# Autodesk Inventor assembly: Robot
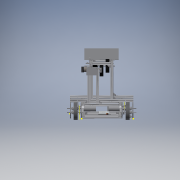
[picture p0: Inventor's stored thumbnail of the model, 180x180]
Saved by Autodesk Inventor 2016 (Build 200138000, 138)
## iProperties
Created: 2016-10-08
Part Number: Robot
Document SubType Name: Assembly
Designer: RoboticsUser
Author: RoboticsUser
## Documents named in this file (17)
- C:\Robotics\CAD\2016-17_CAD\Robot.iam
- C:\Robotics\CAD\2016-17_CAD\WheelAssemblyWFrame.iam
- C:\Robotics\CAD\COTSParts\Bosch Extrusion\Bosch 20x20 9 in.ipt
- C:\Robotics\CAD\COTSParts\Bosch Extrusion\Gusset 20x20 w screws.ipt
- C:\Robotics\CAD\COTSParts\Bosch Extrusion\Bosch 20x20 9 in - Copy.ipt
- C:\Robotics\CAD\COTSParts\Bosch Extrusion\Rexroth-6mmT-Nutm4.ipt
- C:\Robotics\CAD\COTSParts\Bosch Extrusion\Rexroth-GussetwFastenersm4x8.ipt
- C:\Robotics\CAD\COTSParts\Bosch Extrusion\Bosch 20x20 8.937in.ipt
- C:\Robotics\CAD\COTSParts\Bosch Extrusion\Bosch 20x20 9 in actual.ipt
- C:\Robotics\CAD\2016-17_CAD\ParticleLauncher2.0.iam
- C:\Robotics\CAD\2016-17_CAD\BBP.iam
- C:\Robotics\CAD\2016-17_CAD\ElectronicsPlate2.ipt
- C:\Robotics\CAD\COTSParts\ModernRobotics\MRI45-2204_Servo_Controller.ipt
- C:\Robotics\CAD\COTSParts\ModernRobotics\MRI45-2201_Device_Interface.ipt
- C:\Robotics\CAD\2016-17_CAD\Deflecter.ipt
- C:\Robotics\CAD\COTSParts\Bosch Extrusion\Bosch 20x20 16.66 -.ipt
- C:\Robotics\CAD\COTSParts\Actobotics\585 parts\585424.ipt
## Components (55 placed, 16 different names)
1. WheelAssemblyWFrame:1 [sub-assembly] — Mate:1, Insert:4, Insert:5, Insert:6, Flush:29, Mate:55, Flush:37, Flush:42, Flush:83, Mate:144
2. WheelAssemblyWFrame:2 [sub-assembly] — Mate:8, Mate:9, Flush:7, Flush:8, Insert:1, Insert:2, Insert:3, Flush:30, Flush:35, Mate:57, Mate:58, Mate:77, Mate:107, Flush:82, Mate:143, Flush:88, Flush:90, Flush:99
3. Bosch 20x20 9 in:1 — Flush:37, Mate:56, Mate:58, Mate:69, Flush:40, Mate:70, Mate:71, Mate:72, Flush:42, Mate:73, Flush:43, Mate:75, Flush:44, Mate:77
4. Gusset 20x20 w screws:1 — Mate:9, Flush:7, Mate:10
5. Gusset 20x20 w screws:2 — Mate:1
6. Gusset 20x20 w screws:3 — Mate:8
7. Gusset 20x20 w screws:4 — Mate:11, Flush:9
8. Bosch 20x20 9 in:2 — Mate:10, Flush:8, Mate:11, Flush:9, Flush:35, Mate:55
9. Bosch 20x20 9 in - Copy:1 — Mate:33, Flush:25, Flush:28, Flush:30, Flush:31, Mate:44, Flush:34, Mate:52, Mate:53, Mate:131, Mate:142
10. Rexroth-6mmT-Nutm4:1 — Insert:1
11. Rexroth-6mmT-Nutm4:2 — Insert:3, Mate:33, Flush:25
12. Rexroth-6mmT-Nutm4:3 — Insert:2
13. Bosch 20x20 9 in - Copy:2 — Mate:15, Flush:11, Mate:35, Mate:39, Flush:27, Flush:29, Flush:32, Mate:48, Flush:33, Mate:54
14. Rexroth-6mmT-Nutm4:4 — Insert:4
15. Rexroth-6mmT-Nutm4:5 — Insert:5
16. Rexroth-6mmT-Nutm4:6 — Insert:6, Mate:15, Flush:11
17. Bosch 20x20 9 in:3 — Flush:27, Flush:31, Mate:50, Mate:51, Mate:53, Mate:54, Flush:69, Mate:141
18. Bosch 20x20 9 in:4 — Mate:39, Flush:28, Flush:32, Mate:45, Mate:46, Mate:47, Mate:49, Flush:33, Flush:34, Mate:106, Mate:130
19. Gusset 20x20 w screws:5 — Mate:51, Mate:52
20. Gusset 20x20 w screws:6 — Mate:35, Mate:50
21. Gusset 20x20 w screws:7 — Mate:47, Mate:48, Mate:49
22. Gusset 20x20 w screws:8 — Mate:44, Mate:45, Mate:46
23. Rexroth-GussetwFastenersm4x8:4 — Mate:56, Mate:57
24. Gusset 20x20 w screws:11 — Mate:70, Mate:71, Mate:76
25. Gusset 20x20 w screws:12 — Mate:69, Flush:40, Mate:72, Mate:74
26. Bosch 20x20 9 in actual:1 — Mate:73, Flush:43, Mate:74, Flush:66, Mate:104, Flush:68
27. Bosch 20x20 9 in actual:2 — Mate:75, Flush:44, Mate:76, Mate:100, Mate:101, Mate:102, Flush:67, Mate:126
28. Bosch 20x20 8.937in:3 — Mate:149, Flush:91, Mate:150, Mate:153, Flush:105, Flush:106
29. Bosch 20x20 8.937in:4 — Mate:93, Flush:62, Mate:146, Mate:147, Flush:86, Flush:92, Flush:103, Flush:104, Mate:160
30. Gusset 20x20 w screws:13 — Flush:84, Mate:145, Mate:146, Flush:86
31. Gusset 20x20 w screws:14 — Mate:148, Flush:87, Flush:88, Flush:91, Mate:150
32. Bosch 20x20 8.937in:5 — Mate:98, Flush:77, Mate:155, Flush:100, Mate:156, Flush:107, Flush:108
33. Bosch 20x20 8.937in:6 — Mate:96, Flush:64, Mate:158, Flush:102, Mate:159, Flush:109
34. ParticleLauncher2.0:1 [sub-assembly] — Flush:103, Flush:104, Mate:160, Flush:105, Flush:106, Flush:107, Flush:108, Flush:109, Mate:161, Mate:162, Mate:163, Mate:164, Mate:165, Mate:166, Mate:167, Mate:168, Mate:169, Mate:170, Mate:171, Mate:172, Mate:174
35. Gusset 20x20 w screws:17 — Mate:153
36. Gusset 20x20 w screws:18 — Mate:93, Flush:62, Flush:92
37. Gusset 20x20 w screws:19 — Mate:96, Flush:64, Mate:161
38. Gusset 20x20 w screws:20 — Mate:98, Flush:77, Mate:162
39. BBP:1 [sub-assembly] — Mate:100, Mate:101, Flush:66, Mate:103, Mate:105, Mate:126
40. Gusset 20x20 w screws:21 — Mate:104, Mate:105, Flush:68
41. Gusset 20x20 w screws:22 — Mate:102, Mate:103, Flush:67
42. ElectronicsPlate2:1 — Mate:106, Flush:69, Mate:107, Mate:129, Mate:140
43. MRI45-2204_Servo_Controller:1 — Mate:140, Mate:141, Mate:142
44. MRI45-2201_Device_Interface:1 — Mate:129, Mate:130, Mate:131
45. Bosch 20x20 16.66 -:1 — Flush:83, Mate:144, Mate:154, Flush:98, Mate:156, Mate:157, Flush:101, Mate:159
46. Bosch 20x20 16.66 -:4 — Flush:82, Mate:143, Flush:84, Mate:145, Mate:147, Mate:148, Flush:87, Flush:90, Mate:149
47. Gusset 20x20 w screws:23 — Mate:154, Flush:98, Flush:99, Mate:155, Flush:100
48. Gusset 20x20 w screws:26 — Mate:157, Flush:101, Mate:158, Flush:102
49. Deflecter:2 — Mate:173, Flush:110, Mate:174
50. 585424:2 — Insert:7, Insert:8, Mate:167, Mate:173, Flush:110
51. Rexroth-6mmT-Nutm4:7 — Mate:165, Mate:166, Insert:7
52. Rexroth-6mmT-Nutm4:8 — Mate:163, Mate:164, Insert:8
53. Rexroth-6mmT-Nutm4:10 — Mate:168, Mate:169, Insert:10
54. Rexroth-6mmT-Nutm4:11 — Mate:170, Mate:171, Insert:9
55. 585424:3 — Insert:9, Insert:10, Mate:172
## Relationships (139: Mate 81, Flush 48, Insert 10)
- Mate:1: WheelAssemblyWFrame:1 ↔ Gusset 20x20 w screws:2
- Mate:8: WheelAssemblyWFrame:2 ↔ Gusset 20x20 w screws:3
- Mate:9: WheelAssemblyWFrame:2 ↔ Gusset 20x20 w screws:1
- Flush:7: WheelAssemblyWFrame:2 ↔ Gusset 20x20 w screws:1
- Mate:10: Gusset 20x20 w screws:1 ↔ Bosch 20x20 9 in:2
- Flush:8: WheelAssemblyWFrame:2 ↔ Bosch 20x20 9 in:2
- Mate:11: Gusset 20x20 w screws:4 ↔ Bosch 20x20 9 in:2
- Flush:9: Gusset 20x20 w screws:4 ↔ Bosch 20x20 9 in:2
- Insert:1: WheelAssemblyWFrame:2 ↔ Rexroth-6mmT-Nutm4:1
- Insert:2: WheelAssemblyWFrame:2 ↔ Rexroth-6mmT-Nutm4:3
- Insert:3: WheelAssemblyWFrame:2 ↔ Rexroth-6mmT-Nutm4:2
- Insert:4: WheelAssemblyWFrame:1 ↔ Rexroth-6mmT-Nutm4:4
- Insert:5: WheelAssemblyWFrame:1 ↔ Rexroth-6mmT-Nutm4:5
- Insert:6: WheelAssemblyWFrame:1 ↔ Rexroth-6mmT-Nutm4:6
- Mate:15: Bosch 20x20 9 in - Copy:2 ↔ Rexroth-6mmT-Nutm4:6
- Flush:11 (64.77 mm): Bosch 20x20 9 in - Copy:2 ↔ Rexroth-6mmT-Nutm4:6
- Mate:33: Bosch 20x20 9 in - Copy:1 ↔ Rexroth-6mmT-Nutm4:2
- Flush:25 (64.77 mm): Bosch 20x20 9 in - Copy:1 ↔ Rexroth-6mmT-Nutm4:2
- Mate:35: Bosch 20x20 9 in - Copy:2 ↔ Gusset 20x20 w screws:6
- Mate:39: Bosch 20x20 9 in - Copy:2 ↔ Bosch 20x20 9 in:4
- Flush:27: Bosch 20x20 9 in - Copy:2 ↔ Bosch 20x20 9 in:3
- Flush:28: Bosch 20x20 9 in - Copy:1 ↔ Bosch 20x20 9 in:4
- Flush:29 (1.6256 mm): WheelAssemblyWFrame:1 ↔ Bosch 20x20 9 in - Copy:2
- Flush:30 (1.6256 mm): WheelAssemblyWFrame:2 ↔ Bosch 20x20 9 in - Copy:1
- Flush:31 (56.896 mm): Bosch 20x20 9 in - Copy:1 ↔ Bosch 20x20 9 in:3
- Flush:32: Bosch 20x20 9 in - Copy:2 ↔ Bosch 20x20 9 in:4
- Mate:44: Bosch 20x20 9 in - Copy:1 ↔ Gusset 20x20 w screws:8
- Mate:45: Bosch 20x20 9 in:4 ↔ Gusset 20x20 w screws:8
- Mate:46: Bosch 20x20 9 in:4 ↔ Gusset 20x20 w screws:8
- Mate:47: Bosch 20x20 9 in:4 ↔ Gusset 20x20 w screws:7
- Mate:48: Bosch 20x20 9 in - Copy:2 ↔ Gusset 20x20 w screws:7
- Mate:49: Bosch 20x20 9 in:4 ↔ Gusset 20x20 w screws:7
- Flush:33: Bosch 20x20 9 in - Copy:2 ↔ Bosch 20x20 9 in:4
- Flush:34: Bosch 20x20 9 in - Copy:1 ↔ Bosch 20x20 9 in:4
- Mate:50: Bosch 20x20 9 in:3 ↔ Gusset 20x20 w screws:6
- Mate:51: Bosch 20x20 9 in:3 ↔ Gusset 20x20 w screws:5
- Mate:52: Bosch 20x20 9 in - Copy:1 ↔ Gusset 20x20 w screws:5
- Mate:53: Bosch 20x20 9 in - Copy:1 ↔ Bosch 20x20 9 in:3
- Mate:54: Bosch 20x20 9 in - Copy:2 ↔ Bosch 20x20 9 in:3
- Flush:35 (127 mm): WheelAssemblyWFrame:2 ↔ Bosch 20x20 9 in:2
- Mate:55: WheelAssemblyWFrame:1 ↔ Bosch 20x20 9 in:2
- Flush:37: WheelAssemblyWFrame:1 ↔ Bosch 20x20 9 in:1
- Mate:56: Bosch 20x20 9 in:1 ↔ Rexroth-GussetwFastenersm4x8:4
- Mate:57: WheelAssemblyWFrame:2 ↔ Rexroth-GussetwFastenersm4x8:4
- Mate:58: WheelAssemblyWFrame:2 ↔ Bosch 20x20 9 in:1
- Mate:69: Bosch 20x20 9 in:1 ↔ Gusset 20x20 w screws:12
- Flush:40: Bosch 20x20 9 in:1 ↔ Gusset 20x20 w screws:12
- Mate:70: Bosch 20x20 9 in:1 ↔ Gusset 20x20 w screws:11
- Mate:71: Bosch 20x20 9 in:1 ↔ Gusset 20x20 w screws:11
- Mate:72: Bosch 20x20 9 in:1 ↔ Gusset 20x20 w screws:12
- Flush:42: WheelAssemblyWFrame:1 ↔ Bosch 20x20 9 in:1
- Mate:73: Bosch 20x20 9 in:1 ↔ Bosch 20x20 9 in actual:1
- Flush:43: Bosch 20x20 9 in:1 ↔ Bosch 20x20 9 in actual:1
- Mate:74: Gusset 20x20 w screws:12 ↔ Bosch 20x20 9 in actual:1
- Mate:75: Bosch 20x20 9 in:1 ↔ Bosch 20x20 9 in actual:2
- Flush:44: Bosch 20x20 9 in:1 ↔ Bosch 20x20 9 in actual:2
- Mate:76: Gusset 20x20 w screws:11 ↔ Bosch 20x20 9 in actual:2
- Mate:77: WheelAssemblyWFrame:2 ↔ Bosch 20x20 9 in:1
- Mate:93: Bosch 20x20 8.937in:4 ↔ Gusset 20x20 w screws:18
- Flush:62: Bosch 20x20 8.937in:4 ↔ Gusset 20x20 w screws:18
- Mate:96: Bosch 20x20 8.937in:6 ↔ Gusset 20x20 w screws:19
- Flush:64: Bosch 20x20 8.937in:6 ↔ Gusset 20x20 w screws:19
- Mate:98: Bosch 20x20 8.937in:5 ↔ Gusset 20x20 w screws:20
- Mate:100: Bosch 20x20 9 in actual:2 ↔ BBP:1
- Mate:101: Bosch 20x20 9 in actual:2 ↔ BBP:1
- Flush:66: Bosch 20x20 9 in actual:1 ↔ BBP:1
- Mate:102: Bosch 20x20 9 in actual:2 ↔ Gusset 20x20 w screws:22
- Mate:103: BBP:1 ↔ Gusset 20x20 w screws:22
- Flush:67: Bosch 20x20 9 in actual:2 ↔ Gusset 20x20 w screws:22
- Mate:104: Bosch 20x20 9 in actual:1 ↔ Gusset 20x20 w screws:21
- Mate:105: BBP:1 ↔ Gusset 20x20 w screws:21
- Flush:68: Bosch 20x20 9 in actual:1 ↔ Gusset 20x20 w screws:21
- Mate:106: Bosch 20x20 9 in:4 ↔ ElectronicsPlate2:1
- Flush:69: Bosch 20x20 9 in:3 ↔ ElectronicsPlate2:1
- Mate:107: WheelAssemblyWFrame:2 ↔ ElectronicsPlate2:1
- Mate:126: Bosch 20x20 9 in actual:2 ↔ BBP:1
- Mate:129: ElectronicsPlate2:1 ↔ MRI45-2201_Device_Interface:1
- Mate:130: Bosch 20x20 9 in:4 ↔ MRI45-2201_Device_Interface:1
- Mate:131 (76.7969 mm): Bosch 20x20 9 in - Copy:1 ↔ MRI45-2201_Device_Interface:1
- Flush:77: Bosch 20x20 8.937in:5 ↔ Gusset 20x20 w screws:20
- Mate:140: ElectronicsPlate2:1 ↔ MRI45-2204_Servo_Controller:1
- Mate:141: Bosch 20x20 9 in:3 ↔ MRI45-2204_Servo_Controller:1
- Mate:142 (50.8 mm): Bosch 20x20 9 in - Copy:1 ↔ MRI45-2204_Servo_Controller:1
- Flush:82: WheelAssemblyWFrame:2 ↔ Bosch 20x20 16.66 -:4
- Mate:143: WheelAssemblyWFrame:2 ↔ Bosch 20x20 16.66 -:4
- Flush:83: WheelAssemblyWFrame:1 ↔ Bosch 20x20 16.66 -:1
- Mate:144: WheelAssemblyWFrame:1 ↔ Bosch 20x20 16.66 -:1
- Flush:84: Gusset 20x20 w screws:13 ↔ Bosch 20x20 16.66 -:4
- Mate:145: Gusset 20x20 w screws:13 ↔ Bosch 20x20 16.66 -:4
- Mate:146: Bosch 20x20 8.937in:4 ↔ Gusset 20x20 w screws:13
- Mate:147: Bosch 20x20 8.937in:4 ↔ Bosch 20x20 16.66 -:4
- Flush:86: Bosch 20x20 8.937in:4 ↔ Gusset 20x20 w screws:13
- Mate:148: Gusset 20x20 w screws:14 ↔ Bosch 20x20 16.66 -:4
- Flush:87: Gusset 20x20 w screws:14 ↔ Bosch 20x20 16.66 -:4
- Flush:88 (-55.0672 mm): WheelAssemblyWFrame:2 ↔ Gusset 20x20 w screws:14
- Flush:90: WheelAssemblyWFrame:2 ↔ Bosch 20x20 16.66 -:4
- Mate:149: Bosch 20x20 8.937in:3 ↔ Bosch 20x20 16.66 -:4
- Flush:91: Bosch 20x20 8.937in:3 ↔ Gusset 20x20 w screws:14
- Mate:150: Bosch 20x20 8.937in:3 ↔ Gusset 20x20 w screws:14
- Flush:92: Bosch 20x20 8.937in:4 ↔ Gusset 20x20 w screws:18
- Mate:153: Bosch 20x20 8.937in:3 ↔ Gusset 20x20 w screws:17
- Mate:154: Bosch 20x20 16.66 -:1 ↔ Gusset 20x20 w screws:23
- Flush:98: Bosch 20x20 16.66 -:1 ↔ Gusset 20x20 w screws:23
- Flush:99 (-55.0672 mm): WheelAssemblyWFrame:2 ↔ Gusset 20x20 w screws:23
- Mate:155: Bosch 20x20 8.937in:5 ↔ Gusset 20x20 w screws:23
- Flush:100: Bosch 20x20 8.937in:5 ↔ Gusset 20x20 w screws:23
- Mate:156: Bosch 20x20 8.937in:5 ↔ Bosch 20x20 16.66 -:1
- Mate:157: Bosch 20x20 16.66 -:1 ↔ Gusset 20x20 w screws:26
- Flush:101: Bosch 20x20 16.66 -:1 ↔ Gusset 20x20 w screws:26
- Mate:158: Bosch 20x20 8.937in:6 ↔ Gusset 20x20 w screws:26
- Flush:102: Bosch 20x20 8.937in:6 ↔ Gusset 20x20 w screws:26
- Mate:159: Bosch 20x20 8.937in:6 ↔ Bosch 20x20 16.66 -:1
- Flush:103: Bosch 20x20 8.937in:4 ↔ ParticleLauncher2.0:1
- Flush:104: Bosch 20x20 8.937in:4 ↔ ParticleLauncher2.0:1
- Mate:160: Bosch 20x20 8.937in:4 ↔ ParticleLauncher2.0:1
- Flush:105: Bosch 20x20 8.937in:3 ↔ ParticleLauncher2.0:1
- Flush:106: Bosch 20x20 8.937in:3 ↔ ParticleLauncher2.0:1
- Flush:107: Bosch 20x20 8.937in:5 ↔ ParticleLauncher2.0:1
- Flush:108: Bosch 20x20 8.937in:5 ↔ ParticleLauncher2.0:1
- Flush:109: Bosch 20x20 8.937in:6 ↔ ParticleLauncher2.0:1
- Mate:161: ParticleLauncher2.0:1 ↔ Gusset 20x20 w screws:19
- Mate:162: ParticleLauncher2.0:1 ↔ Gusset 20x20 w screws:20
- Mate:163: ParticleLauncher2.0:1 ↔ Rexroth-6mmT-Nutm4:8
- Mate:164: ParticleLauncher2.0:1 ↔ Rexroth-6mmT-Nutm4:8
- Mate:165: ParticleLauncher2.0:1 ↔ Rexroth-6mmT-Nutm4:7
- Mate:166: ParticleLauncher2.0:1 ↔ Rexroth-6mmT-Nutm4:7
- Insert:7: 585424:2 ↔ Rexroth-6mmT-Nutm4:7
- Insert:8: 585424:2 ↔ Rexroth-6mmT-Nutm4:8
- Mate:167 (-165.1 mm): ParticleLauncher2.0:1 ↔ 585424:2
- Mate:168: ParticleLauncher2.0:1 ↔ Rexroth-6mmT-Nutm4:10
- Mate:169: ParticleLauncher2.0:1 ↔ Rexroth-6mmT-Nutm4:10
- Mate:170: ParticleLauncher2.0:1 ↔ Rexroth-6mmT-Nutm4:11
- Mate:171: ParticleLauncher2.0:1 ↔ Rexroth-6mmT-Nutm4:11
- Insert:9: Rexroth-6mmT-Nutm4:11 ↔ 585424:3
- Insert:10: Rexroth-6mmT-Nutm4:10 ↔ 585424:3
- Mate:172 (-165.1 mm): ParticleLauncher2.0:1 ↔ 585424:3
- Mate:173: Deflecter:2 ↔ 585424:2
- Flush:110 (27.1018 mm): Deflecter:2 ↔ 585424:2
- Mate:174: ParticleLauncher2.0:1 ↔ Deflecter:2
